# Autodesk Inventor assembly: Assembly@@
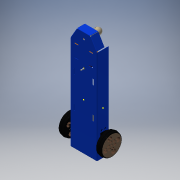
[picture p0: Inventor's stored thumbnail of the model, 180x180]
Saved by Autodesk Inventor 2016 (Build 200138000, 138)
## iProperties
Created: 2016-10-26
Part Number: Assembly@@
Document SubType Name: Assembly
Designer: desirw
Author: desirw
## Documents named in this file (11)
- H:\My Documents\ROBOT\Assembly@@.iam
- H:\My Documents\ROBOT\Wheel.ipt
- H:\My Documents\ROBOT\Ball.ipt
- H:\My Documents\ROBOT\Battery - Copy.ipt
- H:\My Documents\ROBOT\Breadboard.ipt
- H:\My Documents\ROBOT\Castor.ipt
- H:\My Documents\ROBOT\Chassis2.ipt
- H:\My Documents\ROBOT\Motor.ipt
- H:\My Documents\ROBOT\O-RING.ipt
- H:\My Documents\ROBOT\Servo Horn HONK HONK.ipt
- H:\My Documents\ROBOT\Switch.ipt
## Components (14 placed, 10 different names)
1. Wheel:1 — Mate:9, Mate:10, Mate:11, Rigid:5
2. Ball:1 — Mate:13
3. Battery - Copy:1 — Mate:5
4. Breadboard:1 — Mate:1, Mate:2, Mate:3, Mate:4
5. Castor:1 — Rigid:3, Mate:13, Mate:14
6. Chassis2:1 — Mate:1, Mate:2, Mate:3, Mate:4, Mate:5, Rigid:1, Rigid:2, Rigid:3, Mate:12, Mate:14
7. Motor:1 — Rigid:1, Rotational:2
8. O-RING:1 — Rigid:4
9. Servo Horn HONK HONK:1 — Rotational:2, Mate:9, Mate:10, Mate:11
10. Switch:1 — Mate:12
11. Wheel:2 — Mate:6, Mate:7, Mate:8, Rigid:4
12. Motor:2 — Rigid:2, Rotational:1
13. O-RING:2 — Rigid:5
14. Servo Horn HONK HONK:2 — Rotational:1, Mate:6, Mate:7, Mate:8
## Relationships (21: Mate 14, WeldJoint 5, RevoluteJoint 2)
- Mate:1: Breadboard:1 ↔ Chassis2:1
- Mate:2: Breadboard:1 ↔ Chassis2:1
- Mate:3: Breadboard:1 ↔ Chassis2:1
- Mate:4: Breadboard:1 ↔ Chassis2:1
- Mate:5: Battery - Copy:1 ↔ Chassis2:1
- Rigid:1 [WeldJoint]: Chassis2:1 ↔ Motor:1
- Rigid:2 [WeldJoint]: Chassis2:1 ↔ Motor:2
- Rigid:3 [WeldJoint]: Castor:1 ↔ Chassis2:1
- Rotational:1 [RevoluteJoint]: Motor:2 ↔ Servo Horn HONK HONK:2
- Rotational:2 [RevoluteJoint]: Motor:1 ↔ Servo Horn HONK HONK:1
- Mate:6: Wheel:2 ↔ Servo Horn HONK HONK:2
- Mate:7: Wheel:2 ↔ Servo Horn HONK HONK:2
- Mate:8: Wheel:2 ↔ Servo Horn HONK HONK:2
- Mate:9: Wheel:1 ↔ Servo Horn HONK HONK:1
- Mate:10: Wheel:1 ↔ Servo Horn HONK HONK:1
- Mate:11: Wheel:1 ↔ Servo Horn HONK HONK:1
- Mate:12: Chassis2:1 ↔ Switch:1
- Rigid:4 [WeldJoint]: O-RING:1 ↔ Wheel:2
- Rigid:5 [WeldJoint]: Wheel:1 ↔ O-RING:2
- Mate:13: Ball:1 ↔ Castor:1
- Mate:14: Castor:1 ↔ Chassis2:1
